# Autodesk Inventor assembly: cabinet_assembly
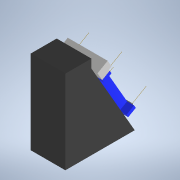
[picture p0: Inventor's stored thumbnail of the model, 180x180]
Saved by Autodesk Inventor 2020 (Build 240168000, 168)
## iProperties
Created: 2021-03-06
Part Number: cabinet_assembly
Document SubType Name: Assembly
Designer: Harry
Author: Harry
## Documents named in this file (3)
- C:\Users\Harry\Documents\hacktheburgh\octocatch\cad\cabinet_assembly.iam
- C:\Users\Harry\Documents\hacktheburgh\octocatch\cad\cabinet.ipt
- C:\Users\Harry\Documents\hacktheburgh\octocatch\cad\main_assembly.iam
## Components (2 placed, 2 different names)
1. cabinet:1 — Mate:1
2. main_assembly:1 [sub-assembly] — Mate:1
## Relationships (1: Mate 1)
- Mate:1: cabinet:1 ↔ main_assembly:1
